# Autodesk Inventor assembly: armTens
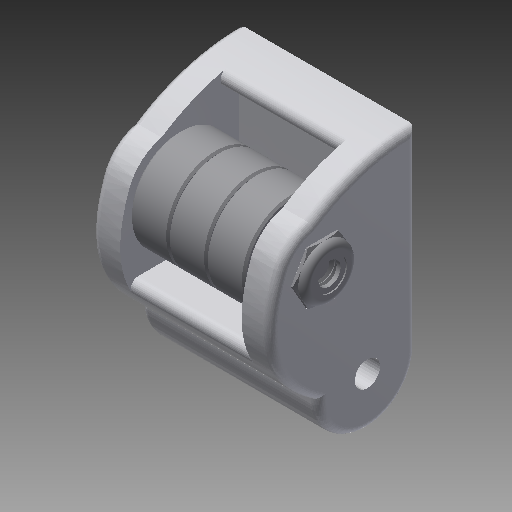
[picture p0: Inventor's stored thumbnail of the model, 512x512]
Saved by Autodesk Inventor 2019 (Build 230136000, 136)
## iProperties
Created: 2020-03-22
Part Number: armTens
Document SubType Name: Assembly
Designer: james
Author: james
## Documents named in this file (5)
- F:\JimsRobot\FIRSTRobots\Design\RBX1-REMIX\arm\armTens.iam
- F:\JimsRobot\FIRSTRobots\Design\RBX1-REMIX\arm\arm_tensioner_qty1.ipt
- F:\JimsRobot\FIRSTRobots\Design\Library\McMaster\Bearings\7804K103_STAINLESS STEEL BALL BEARING 4x13x5.ipt
- F:\JimsRobot\FIRSTRobots\Design\Library\McMaster\SocketScrews\M4-20 91290A168_BLACK-OXIDE CLASS 12.9 SOCKET HEAD CAP SCREW.ipt
- F:\JimsRobot\FIRSTRobots\Design\Library\McMaster\Nuts\M4 94645A101_HIGH-STRENGTH STEEL NYLON-INSERT LOCKNUT.ipt
## Components (6 placed, 4 different names)
1. arm_tensioner_qty1:1 — Mate:5, Mate:6, Mate:7
2. 7804K103_STAINLESS STEEL BALL BEARING 4x13x5:1 — Mate:1, Mate:2, Mate:3
3. 7804K103_STAINLESS STEEL BALL BEARING 4x13x5:2 — Mate:1, Mate:2, Mate:4, Mate:5, Mate:9
4. 7804K103_STAINLESS STEEL BALL BEARING 4x13x5:3 — Mate:3, Mate:4, Mate:6, Mate:8
5. M4-20 91290A168_BLACK-OXIDE CLASS 12.9 SOCKET HEAD CAP SCREW:1 — Mate:7, Mate:8, Mate:10
6. M4 94645A101_HIGH-STRENGTH STEEL NYLON-INSERT LOCKNUT:1 — Mate:9, Mate:10
## Relationships (10: Mate 10)
- Mate:1: 7804K103_STAINLESS STEEL BALL BEARING 4x13x5:1 ↔ 7804K103_STAINLESS STEEL BALL BEARING 4x13x5:2
- Mate:2: 7804K103_STAINLESS STEEL BALL BEARING 4x13x5:1 ↔ 7804K103_STAINLESS STEEL BALL BEARING 4x13x5:2
- Mate:3: 7804K103_STAINLESS STEEL BALL BEARING 4x13x5:1 ↔ 7804K103_STAINLESS STEEL BALL BEARING 4x13x5:3
- Mate:4: 7804K103_STAINLESS STEEL BALL BEARING 4x13x5:2 ↔ 7804K103_STAINLESS STEEL BALL BEARING 4x13x5:3
- Mate:5: arm_tensioner_qty1:1 ↔ 7804K103_STAINLESS STEEL BALL BEARING 4x13x5:2
- Mate:6: arm_tensioner_qty1:1 ↔ 7804K103_STAINLESS STEEL BALL BEARING 4x13x5:3
- Mate:7: arm_tensioner_qty1:1 ↔ M4-20 91290A168_BLACK-OXIDE CLASS 12.9 SOCKET HEAD CAP SCREW:1
- Mate:8: 7804K103_STAINLESS STEEL BALL BEARING 4x13x5:3 ↔ M4-20 91290A168_BLACK-OXIDE CLASS 12.9 SOCKET HEAD CAP SCREW:1
- Mate:9: 7804K103_STAINLESS STEEL BALL BEARING 4x13x5:2 ↔ M4 94645A101_HIGH-STRENGTH STEEL NYLON-INSERT LOCKNUT:1
- Mate:10: M4-20 91290A168_BLACK-OXIDE CLASS 12.9 SOCKET HEAD CAP SCREW:1 ↔ M4 94645A101_HIGH-STRENGTH STEEL NYLON-INSERT LOCKNUT:1
